# Autodesk Inventor assembly: FeederV3
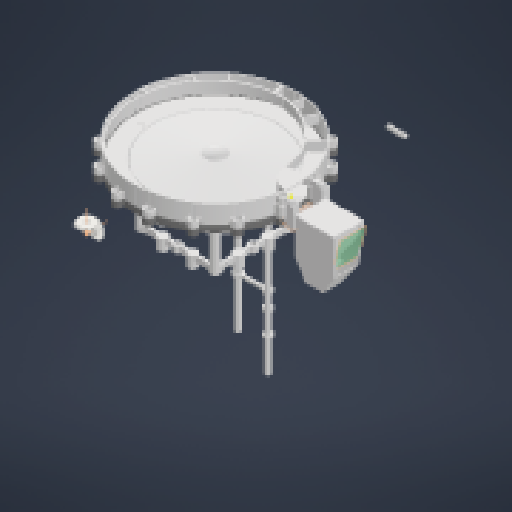
[picture p0: Inventor's stored thumbnail of the model, 512x512]
Saved by Autodesk Inventor 2026 (Build 300175050, 175E)
## iProperties
Created: 2026-03-26
Part Number: FeederV3
Document SubType Name: Assembly
Designer: sniel
Author: sniel
## Documents named in this file (43)
- C:\Users\sniel\OneDrive\SDU\4_Semester\Applied automation\AppliedAutomationProject\feeder\FeederV3.iam
- C:\Users\sniel\OneDrive\SDU\4_Semester\Applied automation\AppliedAutomationProject\feeder\base plate.ipt
- C:\Users\sniel\OneDrive\SDU\4_Semester\Applied automation\AppliedAutomationProject\feeder\outerspinnerV3.ipt
- C:\Users\sniel\OneDrive\SDU\4_Semester\Applied automation\AppliedAutomationProject\feeder\gears1.ipt
- C:\Users\sniel\OneDrive\SDU\4_Semester\Applied automation\AppliedAutomationProject\feeder\FeederV2\Design Accelerator\Spur Gears5.iam
- C:\Users\sniel\OneDrive\SDU\4_Semester\Applied automation\AppliedAutomationProject\feeder\centrer centrifugal spinner.ipt
- C:\Users\sniel\OneDrive\SDU\4_Semester\Applied automation\AppliedAutomationProject\feeder\central axel.ipt
- C:\Users\sniel\OneDrive\SDU\4_Semester\Applied automation\AppliedAutomationProject\feeder\base frame.ipt
- C:\Users\sniel\OneDrive\SDU\4_Semester\Applied automation\AppliedAutomationProject\feeder\moon_gear_V1.ipt
- C:\Users\sniel\OneDrive\SDU\4_Semester\Applied automation\AppliedAutomationProject\feeder\primlock.ipt
- C:\Users\sniel\OneDrive\SDU\4_Semester\Applied automation\AppliedAutomationProject\feeder\outerdisk_pin.ipt
- C:\Users\sniel\OneDrive\SDU\4_Semester\Applied automation\AppliedAutomationProject\feeder\roll_ball_1.ipt
- C:\Users\sniel\OneDrive\SDU\4_Semester\Applied automation\AppliedAutomationProject\feeder\Leg_v1.ipt
- C:\Users\sniel\OneDrive\SDU\4_Semester\Applied automation\AppliedAutomationProject\feeder\main axel.ipt
- C:\Users\sniel\OneDrive\SDU\4_Semester\Applied automation\AppliedAutomationProject\feeder\ServoMotor.ipt
- C:\Users\sniel\OneDrive\SDU\4_Semester\Applied automation\AppliedAutomationProject\feeder\Base_frame_v2.ipt
- C:\Users\sniel\OneDrive\SDU\4_Semester\Applied automation\AppliedAutomationProject\feeder\Metal bearing.ipt
- C:\Users\sniel\OneDrive\SDU\4_Semester\Applied automation\AppliedAutomationProject\feeder\FeederV2\Design Accelerator\Spur Gears11.iam
- C:\Users\sniel\OneDrive\SDU\4_Semester\Applied automation\AppliedAutomationProject\feeder\Central_axel_Gear.ipt
- C:\Users\sniel\OneDrive\SDU\4_Semester\Applied automation\AppliedAutomationProject\feeder\halfAxel.ipt
- C:\Users\sniel\OneDrive\SDU\4_Semester\Applied automation\AppliedAutomationProject\feeder\TopSpinner_steep_angle_V2.ipt
- C:\Users\sniel\OneDrive\SDU\4_Semester\Applied automation\AppliedAutomationProject\feeder\STEP\45angleBase.ipt
- C:\Users\sniel\OneDrive\SDU\4_Semester\Applied automation\AppliedAutomationProject\feeder\FeederV2\Design Accelerator\Bevel Gears1.iam
- C:\Users\sniel\OneDrive\SDU\4_Semester\Applied automation\AppliedAutomationProject\feeder\FeederV2\Design Accelerator\Bevel Gears2.iam
- C:\Users\sniel\OneDrive\SDU\4_Semester\Applied automation\AppliedAutomationProject\feeder\FeederV2\Design Accelerator\Bevel Gears3.iam
- C:\Users\sniel\OneDrive\SDU\4_Semester\Applied automation\AppliedAutomationProject\feeder\long_axel.ipt
- C:\Users\sniel\OneDrive\SDU\4_Semester\Applied automation\AppliedAutomationProject\feeder\filter1.ipt
- C:\Users\sniel\OneDrive\SDU\4_Semester\Applied automation\AppliedAutomationProject\feeder\STEP\LegV2.ipt
- C:\Users\sniel\OneDrive\SDU\4_Semester\Applied automation\AppliedAutomationProject\feeder\STEP\Leg_rod.ipt
- C:\Users\sniel\OneDrive\SDU\4_Semester\Applied automation\AppliedAutomationProject\feeder\STEP\wall_pin.ipt
- C:\Users\sniel\OneDrive\SDU\4_Semester\Applied automation\AppliedAutomationProject\feeder\STEP\HalfFilterwall.ipt
- C:\Users\sniel\OneDrive\SDU\4_Semester\Applied automation\AppliedAutomationProject\feeder\STEP\HalfFilterWall2.ipt
- C:\Users\sniel\OneDrive\SDU\4_Semester\Applied automation\AppliedAutomationProject\feeder\trayFeeder\HalfFilterwall3.ipt
- C:\Users\sniel\OneDrive\SDU\4_Semester\Applied automation\AppliedAutomationProject\feeder\outerspinner assembled.iam
- C:\Users\sniel\OneDrive\SDU\4_Semester\Applied automation\AppliedAutomationProject\feeder\capflipper.iam
- C:\Users\sniel\OneDrive\SDU\4_Semester\Applied automation\AppliedAutomationProject\feeder\STEP\Wall v2\HalfFilterwall2.5.ipt
- C:\Users\sniel\OneDrive\SDU\4_Semester\Applied automation\AppliedAutomationProject\feeder\STEP\Wall v2\center_disk.ipt
- C:\Users\sniel\OneDrive\SDU\4_Semester\Applied automation\AppliedAutomationProject\feeder\STEP\Wall v2\Central_spinner_cap.ipt
- C:\Users\sniel\OneDrive\SDU\4_Semester\Applied automation\AppliedAutomationProject\feeder\Axel_connector.ipt
- C:\Users\sniel\OneDrive\SDU\4_Semester\Applied automation\AppliedAutomationProject\feeder\Very_long_axel.ipt
- C:\Users\sniel\OneDrive\SDU\4_Semester\Applied automation\AppliedAutomationProject\feeder\Pillar.ipt
- C:\Users\sniel\OneDrive\SDU\4_Semester\Applied automation\AppliedAutomationProject\feeder\Pillar_side.ipt
- C:\Users\sniel\OneDrive\SDU\4_Semester\Applied automation\AppliedAutomationProject\feeder\Pillar_corner_v2.ipt
## Components (57 placed, 39 different names)
1. base plate:1
2. outerspinnerV3:1 — Mate:1, Mate:2, Mate:3, Mate:4, Flush:2, Mate:6
3. gears1:1 — Mate:3
4. Spur Gears:4 [sub-assembly] — Mate:1, Mate:2
5. centrer centrifugal spinner:1 — Mate:4, Flush:1
6. central axel:1 — Flush:1, Mate:5, Flush:4
7. base frame:1 — Mate:5, Flush:2, Mate:6, Mate:7, Mate:8, Mate:9, Mate:11, Mate:12, Mate:13, Mate:14
8. moon_gear_V1:1 — Mate:7, Mate:8, Mate:10, Flush:3
9. moon_gear_V1:2 — Mate:9, Mate:11
10. primlock:1 — Mate:10, Flush:3
11. outerdisk_pin:1 — Mate:12
12. roll_ball_1:1
13. Leg_v1:1 — Mate:13, Mate:14
14. main axel:1 — Flush:4
15. ServoMotor:1 — Mate:15, Mate:16, Mate:17
16. Base_frame_v2:1 — Mate:15, Mate:16, Mate:17, Mate:19, Mate:20, Mate:24, Mate:26, Flush:9, Flush:10, Mate:28, Flush:13, Mate:29, Mate:75, Mate:76, Mate:77, Mate:90, Mate:91, Mate:92
17. Spur Gears:5 [sub-assembly]
18. Central_axel_Gear:1 — Mate:19, Mate:20, Mate:79, Flush:21
19. Metal bearing:2 — Mate:24, Mate:25
20. halfAxel:1 — Mate:25
21. TopSpinner_steep_angle_V2:1
22. Base_frame_v2:2 — Mate:26, Flush:9, Flush:10, Mate:32, Flush:15, Mate:71, Mate:72, Mate:83, Mate:87, Mate:88, Mate:89
23. Base_frame_v2:3 — Mate:68, Mate:69, Mate:70, Mate:78
24. Base_frame_v2:4 — Mate:28, Flush:13, Mate:29, Mate:67, Flush:20
25. 45angleBase:1
26. Metal bearing:3 — Mate:32, Flush:15, Mate:33, Mate:34, Mate:93
27. Bevel Gears:1 [sub-assembly]
28. Bevel Gears:2 [sub-assembly]
29. Bevel Gears:3 [sub-assembly]
30. halfAxel:2 — Mate:33, Mate:34
31. Metal bearing:4
32. long_axel:1
33. filter1:1
34. LegV2:1 — Mate:67, Flush:17, Mate:84
35. LegV2:2 — Mate:68, Mate:69, Mate:70, Flush:18
36. Leg_rod:1 — Flush:17, Flush:18, Flush:23, Mate:99, Mate:100
37. wall_pin:1 — Mate:71, Mate:72
38. HalfFilterwall:1 — Mate:75, Mate:76, Mate:77
39. HalfFilterWall2:1 — Mate:78, Mate:81
40. HalfFilterwall3:1 — Flush:20, Mate:80, Mate:82
41. outerspinner assembled:1 [sub-assembly] — Mate:79
42. capflipper:1 [sub-assembly] — Mate:80, Mate:81, Mate:82
43. HalfFilterwall2.5:1 — Mate:83
44. center_disk:1 — Flush:21, Flush:22
45. Central_spinner_cap:1 — Flush:22
46. Leg_rod:2 — Flush:23, Mate:84
47. LegV2:4 — Mate:87, Mate:88, Mate:89, Flush:24, Flush:25
48. LegV2:5 — Mate:90, Mate:91, Mate:92
49. Leg_rod:3 — Flush:24
50. Leg_rod:4 — Flush:25, Mate:94, Mate:95, Mate:96, Mate:97, Mate:98
51. Axel_connector:1 — Mate:93
52. Very_long_axel:1 — Mate:94
53. Pillar:1 — Mate:95, Mate:96, Mate:102
54. Pillar:2 — Mate:99, Mate:100
55. Pillar:3 — Mate:97, Mate:98, Mate:101, Mate:103
56. Pillar_side:1 — Mate:101, Mate:102
57. Pillar_corner_v2:1 — Mate:103
## Relationships (79: Mate 61, Flush 18)
- Mate:1: outerspinnerV3:1 ↔ Spur Gears:4
- Mate:2: outerspinnerV3:1 ↔ Spur Gears:4
- Mate:3: outerspinnerV3:1 ↔ gears1:1
- Mate:4: outerspinnerV3:1 ↔ centrer centrifugal spinner:1
- Flush:1: centrer centrifugal spinner:1 ↔ central axel:1
- Mate:5: central axel:1 ↔ base frame:1
- Flush:2: outerspinnerV3:1 ↔ base frame:1
- Mate:6: outerspinnerV3:1 ↔ base frame:1
- Mate:7: base frame:1 ↔ moon_gear_V1:1
- Mate:8: base frame:1 ↔ moon_gear_V1:1
- Mate:9: base frame:1 ↔ moon_gear_V1:2
- Mate:10: moon_gear_V1:1 ↔ primlock:1
- Flush:3: moon_gear_V1:1 ↔ primlock:1
- Mate:11: base frame:1 ↔ moon_gear_V1:2
- Mate:12: base frame:1 ↔ outerdisk_pin:1
- Mate:13: base frame:1 ↔ Leg_v1:1
- Mate:14: base frame:1 ↔ Leg_v1:1
- Flush:4: central axel:1 ↔ main axel:1
- Mate:15: ServoMotor:1 ↔ Base_frame_v2:1
- Mate:16: ServoMotor:1 ↔ Base_frame_v2:1
- Mate:17: ServoMotor:1 ↔ Base_frame_v2:1
- Mate:19: Base_frame_v2:1 ↔ Central_axel_Gear:1
- Mate:20 (1 mm): Base_frame_v2:1 ↔ Central_axel_Gear:1
- Mate:24: Base_frame_v2:1 ↔ Metal bearing:2
- Mate:25: Metal bearing:2 ↔ halfAxel:1
- Mate:26: Base_frame_v2:1 ↔ Base_frame_v2:2
- Flush:9: Base_frame_v2:1 ↔ Base_frame_v2:2
- Flush:10: Base_frame_v2:1 ↔ Base_frame_v2:2
- [Mate]: Base_frame_v2:3 ↔ Base_frame_v2:4
- [Flush]: Base_frame_v2:3 ↔ Base_frame_v2:4
- [Flush]: Base_frame_v2:3 ↔ Base_frame_v2:4
- Mate:28: Base_frame_v2:1 ↔ Base_frame_v2:4
- Flush:13: Base_frame_v2:1 ↔ Base_frame_v2:4
- Mate:29: Base_frame_v2:1 ↔ Base_frame_v2:4
- Mate:32: Base_frame_v2:2 ↔ Metal bearing:3
- Flush:15: Base_frame_v2:2 ↔ Metal bearing:3
- Mate:33: Metal bearing:3 ↔ halfAxel:2
- Mate:34: Metal bearing:3 ↔ halfAxel:2
- Mate:67: Base_frame_v2:4 ↔ LegV2:1
- Mate:68: Base_frame_v2:3 ↔ LegV2:2
- Mate:69: Base_frame_v2:3 ↔ LegV2:2
- Mate:70: Base_frame_v2:3 ↔ LegV2:2
- Flush:17: LegV2:1 ↔ Leg_rod:1
- Flush:18: LegV2:2 ↔ Leg_rod:1
- Mate:71: Base_frame_v2:2 ↔ wall_pin:1
- Mate:72: Base_frame_v2:2 ↔ wall_pin:1
- Mate:75: Base_frame_v2:1 ↔ HalfFilterwall:1
- Mate:76 (1 mm): Base_frame_v2:1 ↔ HalfFilterwall:1
- Mate:77: Base_frame_v2:1 ↔ HalfFilterwall:1
- Mate:78 (2 mm): Base_frame_v2:3 ↔ HalfFilterWall2:1
- Flush:20: Base_frame_v2:4 ↔ HalfFilterwall3:1
- Mate:79: Central_axel_Gear:1 ↔ outerspinner assembled:1
- Mate:80: HalfFilterwall3:1 ↔ capflipper:1
- Mate:81: HalfFilterWall2:1 ↔ capflipper:1
- Mate:82 (2 mm): HalfFilterwall3:1 ↔ capflipper:1
- Mate:83 (2 mm): Base_frame_v2:2 ↔ HalfFilterwall2.5:1
- Flush:21: Central_axel_Gear:1 ↔ center_disk:1
- Flush:22: center_disk:1 ↔ Central_spinner_cap:1
- Flush:23: Leg_rod:1 ↔ Leg_rod:2
- Mate:84: LegV2:1 ↔ Leg_rod:2
- Mate:87: Base_frame_v2:2 ↔ LegV2:4
- Mate:88: Base_frame_v2:2 ↔ LegV2:4
- Mate:89: Base_frame_v2:2 ↔ LegV2:4
- Mate:90: Base_frame_v2:1 ↔ LegV2:5
- Mate:91: Base_frame_v2:1 ↔ LegV2:5
- Mate:92: Base_frame_v2:1 ↔ LegV2:5
- Flush:24: LegV2:4 ↔ Leg_rod:3
- Flush:25: LegV2:4 ↔ Leg_rod:4
- Mate:93: Metal bearing:3 ↔ Axel_connector:1
- Mate:94: Leg_rod:4 ↔ Very_long_axel:1
- Mate:95: Leg_rod:4 ↔ Pillar:1
- Mate:96: Leg_rod:4 ↔ Pillar:1
- Mate:97: Leg_rod:4 ↔ Pillar:3
- Mate:98: Leg_rod:4 ↔ Pillar:3
- Mate:99: Leg_rod:1 ↔ Pillar:2
- Mate:100: Leg_rod:1 ↔ Pillar:2
- Mate:101: Pillar:3 ↔ Pillar_side:1
- Mate:102: Pillar:1 ↔ Pillar_side:1
- Mate:103: Pillar:3 ↔ Pillar_corner_v2:1
## Named parameters: d53_d52 = 0 mm, d54_d50 = 0 mm, d55_d51 = 0 mm
